# Autodesk Inventor assembly: board_box_bar_holder
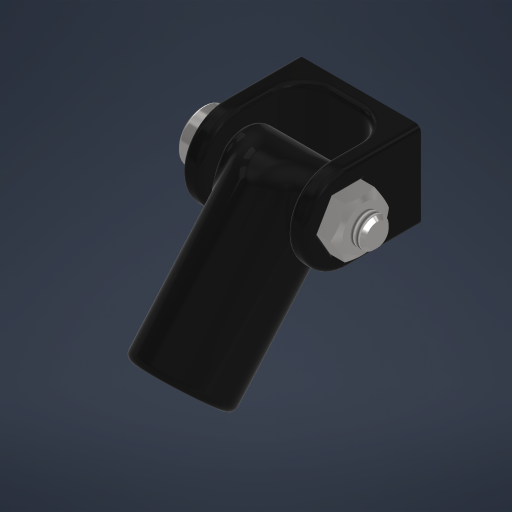
[picture p0: Inventor's stored thumbnail of the model, 512x512]
Saved by Autodesk Inventor 2023 (Build 270158030, 158C)
## iProperties
Created: 2022-07-17
Part Number: board_box_bar_holder
Document SubType Name: Assembly
Designer: Norbert Ligas
Author: Norbert Ligas
## Documents named in this file (5)
- C:\Users\norbe\Repozytoria\NormalMapScanner\3D_modeling\construction\parts\board_box\board_box_bar_holder.iam
- C:\Users\norbe\Repozytoria\NormalMapScanner\3D_modeling\construction\parts\board_box\bar_holder.ipt
- C:\Users\norbe\Repozytoria\NormalMapScanner\3D_modeling\construction\parts\board_box\board_box_holder.ipt
- C:\Users\norbe\OneDrive\Dokumenty\Inventor\Content Center Files\R2023\en-US\ISO 4762(2)\ISO 4762 - M4 x 20ISO.ipt
- C:\Users\norbe\OneDrive\Dokumenty\Inventor\Content Center Files\R2023\en-US\ISO 4032(2)\ISO 4032 - M4 - ISO.ipt
## Components (4 placed, 4 different names)
1. bar_holder:1 — Cylindrical:1, Mate:2, Mate:5
2. board_box_holder:1 — Mate:1, Angle:1, Angle:2, Cylindrical:1, Mate:2, Mate:3, Mate:4, Mate:6, Mate:7
3. ISO 4762 M4 x 20:1 — Mate:5, Mate:6
4. ISO 4032 M4:1 — Mate:3, Mate:4, Mate:7
## Relationships (10: Mate 7, Angle 2, CylindricalJoint 1)
- Mate:1: board_box_holder:1
- Angle:1 (180 deg): board_box_holder:1
- Angle:2 (180 deg): board_box_holder:1
- Cylindrical:1: bar_holder:1 ↔ board_box_holder:1
- Mate:2: bar_holder:1 ↔ board_box_holder:1
- Mate:3: board_box_holder:1 ↔ ISO 4032 M4:1
- Mate:4: board_box_holder:1 ↔ ISO 4032 M4:1
- Mate:5: bar_holder:1 ↔ ISO 4762 M4 x 20:1
- Mate:6: board_box_holder:1 ↔ ISO 4762 M4 x 20:1
- Mate:7: board_box_holder:1 ↔ ISO 4032 M4:1
## Named parameters: bar_holder_bar_diameter = 8 mm, bar_holder_wall_thickness = 2 mm, bar_holder_holder_depth = 20 mm, bar_holder_holder_length = 22 mm, bar_holder_screw_diameter = 4 mm, bar_holder_screw_to_bar_distance = 0.5 mm, bar_connector_width = 2.5 mm, bar_connector_screw_depth = 1 mm, bar_connector_bar_holder_width = 12 mm, bar_connector_length_from_screw_center_to_edge = 6 mm, bar_connector_length_from_screw_center_to_box = 8 mm
